# Autodesk Inventor assembly: 草图
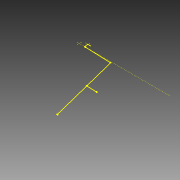
[picture p0: Inventor's stored thumbnail of the model, 180x180]
Saved by Autodesk Inventor 2013 (Build 170138000, 138)
## iProperties
Created: 2012-05-06
Part Number: 草图
Document SubType Name: Assembly
Designer: Zhensheng
Author: Zhensheng
## Documents named in this file (8)
- E:\inventor\牛头刨床概念设计\草图.iam
- E:\inventor\牛头刨床概念设计\草图.ipt
- E:\inventor\牛头刨床概念设计\曲柄.ipt
- E:\inventor\牛头刨床概念设计\摇杆.ipt
- E:\inventor\牛头刨床概念设计\滑块.ipt
- E:\inventor\牛头刨床概念设计\连杆.ipt
- E:\inventor\牛头刨床概念设计\机架one.iam
- E:\inventor\牛头刨床概念设计\导路.ipt
## Components (8 placed, 7 different names)
1. 草图:1
2. 曲柄:1 — 配合:1, 配合:6
3. 摇杆:1 — 配合:2, 配合:3, 配合:7
4. 滑块:1 — 配合:1, 配合:2
5. 连杆:1 — 配合:3, 配合:4
6. 机架one:1 [sub-assembly] — 配合:6, 配合:7
7. 滑块:2 — 配合:4, 配合:5
8. 导路:1 — 配合:5
## Relationships (14: Composite 7, Mate 7)
- [Composite]: 草图:1 ↔ 曲柄:1
- [Composite]: 草图:1 ↔ 摇杆:1
- [Composite]: 草图:1 ↔ 滑块:1
- [Composite]: 草图:1 ↔ 连杆:1
- [Composite]: 草图:1 ↔ 机架one:1
- [Composite]: 草图:1 ↔ 滑块:2
- [Composite]: 草图:1 ↔ 导路:1
- 配合:1 [Mate]: 曲柄:1 ↔ 滑块:1
- 配合:2 [Mate]: 摇杆:1 ↔ 滑块:1
- 配合:3 [Mate]: 摇杆:1 ↔ 连杆:1
- 配合:4 [Mate]: 连杆:1 ↔ 滑块:2
- 配合:5 [Mate]: 滑块:2 ↔ 导路:1
- 配合:6 [Mate]: 曲柄:1 ↔ 机架one:1
- 配合:7 [Mate]: 摇杆:1 ↔ 机架one:1
